# Autodesk Inventor assembly: +XPanel
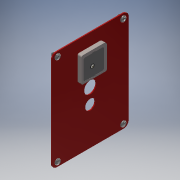
[picture p0: Inventor's stored thumbnail of the model, 180x180]
Saved by Autodesk Inventor 2018 (Build 220112000, 112)
## iProperties
Created: 2018-07-05
Part Number: +XPanel
Document SubType Name: Assembly
Designer: Bradley
Author: Bradley
## Documents named in this file (4)
- D:\Users\Bradley\Documents\CougsInSpace\CougSat1-Hardware\CougSat1-AvionicBoard\CADModel\Native\+XPanel.iam
- D:\Users\Bradley\Documents\CougsInSpace\CougSat1-Hardware\CougSat1-AvionicBoard\CADModel\Native\+XPanel_PCB.ipt
- D:\Users\Bradley\Documents\CougsInSpace\Resources\ComponentModels\Electronics\Antenna_GPSPatch.ipt
- D:\Users\Bradley\Documents\CougsInSpace\Resources\ComponentModels\Fasteners\Bolt_M3x0.35_5mm_BH.ipt
## Components (6 placed, 3 different names)
1. +XPanel_PCB:1 — Insert:1, Insert:2, Insert:3, Insert:4, Insert:5
2. Antenna_GPSPatch:1 — Flush:1, Insert:1
3. Bolt_M3x0.35_5mm_BH:1 — Insert:2
4. Bolt_M3x0.35_5mm_BH:2 — Insert:3
5. Bolt_M3x0.35_5mm_BH:3 — Insert:4
6. Bolt_M3x0.35_5mm_BH:4 — Insert:5
## Relationships (6: Insert 5, Flush 1)
- Flush:1: Antenna_GPSPatch:1
- Insert:1: +XPanel_PCB:1 ↔ Antenna_GPSPatch:1
- Insert:2: +XPanel_PCB:1 ↔ Bolt_M3x0.35_5mm_BH:1
- Insert:3: +XPanel_PCB:1 ↔ Bolt_M3x0.35_5mm_BH:2
- Insert:4: +XPanel_PCB:1 ↔ Bolt_M3x0.35_5mm_BH:3
- Insert:5: +XPanel_PCB:1 ↔ Bolt_M3x0.35_5mm_BH:4
